# Autodesk Inventor assembly: Bumper Assembly
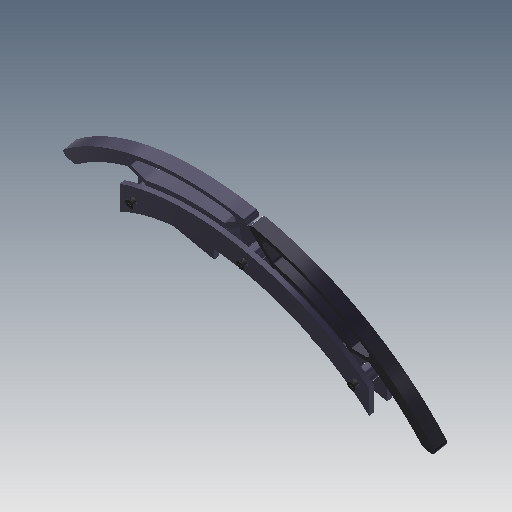
[picture p0: Inventor's stored thumbnail of the model, 512x512]
Saved by Autodesk Inventor 2017 (Build 210142000, 142)
## iProperties
Created: 2017-05-08
Part Number: Bumper Assembly
Document SubType Name: Assembly
Designer: zallen
Author: zallen
## Documents named in this file (12)
- C:\Users\zallen\Documents\GitHub\cr-laundry-robot\src\Base\Bumper Assembly\Bumper Assembly.iam
- C:\Users\zallen\Documents\GitHub\cr-laundry-robot\src\Base\Bumper Assembly\Bumper.ipt
- C:\Users\zallen\Documents\GitHub\cr-laundry-robot\src\Base\Bumper Assembly\Base.ipt
- C:\Users\zallen\Documents\GitHub\cr-laundry-robot\lib\Microswitch\botonera.iam
- C:\Users\zallen\Documents\GitHub\cr-laundry-robot\src\Base\Bumper Assembly\Bumper Assembly\Design Accelerator\Bolted Connection1.iam
- C:\Users\zallen\Documents\GitHub\cr-laundry-robot\src\Base\Bumper Assembly\Bumper Assembly\Design Accelerator\Bolted Connection2.iam
- C:\Users\zallen\Documents\GitHub\cr-laundry-robot\src\Base\Bumper Assembly\Bumper Assembly\Design Accelerator\Bolted Connection5.iam
- C:\Users\zallen\Documents\GitHub\cr-laundry-robot\src\Base\Bumper Assembly\Bumper Assembly\Design Accelerator\Bolted Connection6.iam
- C:\Users\zallen\Documents\GitHub\cr-laundry-robot\src\Base\Bumper Assembly\BaseCover.ipt
- C:\Users\zallen\Documents\GitHub\cr-laundry-robot\src\Base\Bumper Assembly\Bumper Assembly\Design Accelerator\Bolted Connection7.iam
- C:\Users\zallen\Documents\GitHub\cr-laundry-robot\src\Base\Bumper Assembly\Bumper Assembly\Design Accelerator\Bolted Connection8.iam
- C:\Users\zallen\Documents\GitHub\cr-laundry-robot\src\Base\Bumper Assembly\Bumper Assembly\Design Accelerator\Bolted Connection9.iam
## Components (13 placed, 5 different names)
1. Bumper:1 — Mate:5, Mate:36
2. Bumper:2 — Mate:3, Mate:4
3. Base:1 — Mate:3, Mate:4, Mate:5, Mate:8, Mate:17, Mate:18, Mate:19, Mate:20, Mate:21, Mate:26, Mate:27, Mate:28, Mate:29, Mate:31, Mate:33, Mate:35, Mate:36
4. botonera:1 [sub-assembly] — Mate:8, Mate:13, Mate:14, Mate:15, Mate:16, Mate:20, Mate:21
5. botonera:2 [sub-assembly] — Mate:17, Mate:18, Mate:19, Mate:22, Mate:23, Mate:24, Mate:25
6. Bolted Connection:1 [sub-assembly] — Mate:13, Mate:14
7. Bolted Connection:2 [sub-assembly] — Mate:15, Mate:16
8. Bolted Connection:3 [sub-assembly] — Mate:22, Mate:23
9. Bolted Connection:4 [sub-assembly] — Mate:24, Mate:25
10. BaseCover:1 — Mate:26, Mate:27, Mate:28, Mate:29, Mate:30, Mate:32, Mate:34
11. Bolted Connection:5 [sub-assembly] — Mate:30, Mate:31
12. Bolted Connection:6 [sub-assembly] — Mate:32, Mate:33
13. Bolted Connection:7 [sub-assembly] — Mate:34, Mate:35
## Relationships (28: Mate 28)
- Mate:3: Bumper:2 ↔ Base:1
- Mate:4: Bumper:2 ↔ Base:1
- Mate:5: Bumper:1 ↔ Base:1
- Mate:8: Base:1 ↔ botonera:1
- Mate:13: botonera:1 ↔ Bolted Connection:1
- Mate:14: botonera:1 ↔ Bolted Connection:1
- Mate:15: botonera:1 ↔ Bolted Connection:2
- Mate:16: botonera:1 ↔ Bolted Connection:2
- Mate:17: Base:1 ↔ botonera:2
- Mate:18: Base:1 ↔ botonera:2
- Mate:19: Base:1 ↔ botonera:2
- Mate:20: Base:1 ↔ botonera:1
- Mate:21: Base:1 ↔ botonera:1
- Mate:22: botonera:2 ↔ Bolted Connection:3
- Mate:23: botonera:2 ↔ Bolted Connection:3
- Mate:24: botonera:2 ↔ Bolted Connection:4
- Mate:25: botonera:2 ↔ Bolted Connection:4
- Mate:26: Base:1 ↔ BaseCover:1
- Mate:27: Base:1 ↔ BaseCover:1
- Mate:28: Base:1 ↔ BaseCover:1
- Mate:29: Base:1 ↔ BaseCover:1
- Mate:30: BaseCover:1 ↔ Bolted Connection:5
- Mate:31: Base:1 ↔ Bolted Connection:5
- Mate:32: BaseCover:1 ↔ Bolted Connection:6
- Mate:33: Base:1 ↔ Bolted Connection:6
- Mate:34: BaseCover:1 ↔ Bolted Connection:7
- Mate:35: Base:1 ↔ Bolted Connection:7
- Mate:36: Bumper:1 ↔ Base:1
